# Autodesk Inventor assembly: Tower Assembly
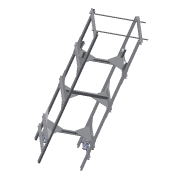
[picture p0: Inventor's stored thumbnail of the model, 180x180]
Saved by Autodesk Inventor 2015 (Build 190159000, 159)
## iProperties
Created: 2015-01-24
Part Number: Tower Assembly
Document SubType Name: Assembly
Designer: Peter
Author: Peter
## Documents named in this file (13)
- C:\Users\Noah\Desktop\FIRST-Team-1719-CAD-Team\2015 Robot CAD\Lifter Super Structure\Tower\Tower Assembly.iam
- C:\Users\Noah\Desktop\FIRST-Team-1719-CAD-Team\2015 Robot CAD\Lifter Super Structure\Tower\Side-Towers Assemblies\Left Side Tower Assembly.iam
- C:\Users\Noah\Desktop\FIRST-Team-1719-CAD-Team\2015 Robot CAD\Lifter Super Structure\Tower\Side-Towers Assemblies\Right Side Tower Assembly.iam
- C:\Users\Noah\Desktop\FIRST-Team-1719-CAD-Team\2015 Robot CAD\Lifter Super Structure\Tower\H-Shaped-Assembly\H-Shaped-Assembly.iam
- C:\Users\Noah\Desktop\FIRST-Team-1719-CAD-Team\2015 Robot CAD\Lifter Super Structure\Tower\Side-Towers Assemblies\Right Side Tower Assembly_MIR.iam
- C:\Users\Noah\Desktop\FIRST-Team-1719-CAD-Team\2015 Robot CAD\Lifter Super Structure\Tower\Side-Towers Assemblies\Left Side Tower Assembly_MIR.iam
- C:\Users\Noah\Desktop\FIRST-Team-1719-CAD-Team\2015 Robot CAD\Lifter Super Structure\Tower\Elevator Motor Assembly\Elevator Motor Assembly_MIR1.iam
- C:\Users\Noah\Desktop\FIRST-Team-1719-CAD-Team\2015 Robot CAD\Lifter Super Structure\Tower\Chain Tension\Chain Tension - L Bracket - Base.ipt
- C:\Users\Noah\Desktop\FIRST-Team-1719-CAD-Team\2015 Robot CAD\Lifter Super Structure\Tower\Chain Tension\Chain Tension - L Bracket.ipt
- C:\Users\Noah\Desktop\FIRST-Team-1719-CAD-Team\2015 Robot CAD\Lifter Super Structure\Tower\Chain Tension\pulley  pinion 1 in 16T 615378 mod1.ipt
- C:\Users\Noah\Desktop\FIRST-Team-1719-CAD-Team\2015 Robot CAD\Lifter Super Structure\Tower\H-Shaped-Assembly\Horizontal-Unistrut-Tower-Connector-15 w holes.ipt
- C:\Users\Noah\Desktop\FIRST-Team-1719-CAD-Team\2015 Robot CAD\Lifter Super Structure\Tower\Top Assembly\Tower connecter.ipt
- C:\Users\Noah\Desktop\FIRST-Team-1719-CAD-Team\2015 Robot CAD\Lifter Super Structure\Tower\Top Assembly\Tower shaft collar bearing.ipt
## Components (29 placed, 12 different names)
1. Right Side Tower Assembly:1 [sub-assembly] — Flush:9, Mate:5, Symmetry:1, Mate:10, Mate:17, Flush:19, Flush:20, Mate:30
2. Left Side Tower Assembly:1 [sub-assembly] — Mate:3, Mate:4, Flush:5, Flush:6, Flush:7, Flush:8, Flush:10, Mate:8, Mate:16, Flush:17, Flush:18, Flush:29
3. H-Shaped-Assembly:5 [sub-assembly] — Mate:3, Flush:5, Flush:8, Mate:7, Flush:13, Mate:9, Flush:14, Mate:11, Mate:12, Flush:15, Flush:16
4. H-Shaped-Assembly:6 [sub-assembly] — Mate:4, Flush:6, Flush:7, Angle:1, Angle:30
5. H-Shaped-Assembly:7 [sub-assembly] — Flush:9, Mate:5, Flush:10
6. Right Side Tower Assembly_MIR:1 [sub-assembly] — Symmetry:1, Mate:15, Flush:23, Flush:24
7. Left Side Tower Assembly_MIR:1 [sub-assembly] — Mate:13, Mate:14, Mate:18, Flush:21, Flush:22, Mate:29, Flush:27, Flush:28
8. Chain Tension - L Bracket - Base:1 — Mate:11, Mate:14, Flush:16, Insert:4
9. Chain Tension - L Bracket - Base:2 — Mate:12, Mate:13, Flush:15, Insert:3, Mate:15
10. Chain Tension - L Bracket - Base:3 — Mate:9, Flush:14, Mate:10, Insert:1
11. Chain Tension - L Bracket - Base:4 — Mate:7, Flush:13, Mate:8, Insert:2
12. Chain Tension - L Bracket:1 — Insert:1, Insert:5
13. Chain Tension - L Bracket:2 — Insert:4, Insert:8
14. Chain Tension - L Bracket:3 — Insert:2, Insert:6
15. Chain Tension - L Bracket:4 — Insert:3, Insert:7
16. pulley  pinion 1 in 16T 615378 mod1:1 — Insert:5
17. pulley  pinion 1 in 16T 615378 mod1:2 — Insert:6
18. pulley  pinion 1 in 16T 615378 mod1:3 — Insert:8
19. pulley  pinion 1 in 16T 615378 mod1:4 — Insert:7
20. Horizontal-Unistrut-Tower-Connector-15 w holes:1 — Mate:18, Flush:21, Flush:22, Flush:23, Flush:24, Flush:25, Mate:23, Mate:28
21. Horizontal-Unistrut-Tower-Connector-15 w holes:2 — Mate:16, Flush:17, Flush:18, Mate:17, Flush:19, Flush:20, Mate:20, Mate:21, Flush:26, Mate:25, Mate:26
22. Tower connecter:1 — Flush:25, Mate:19, Mate:22
23. Tower connecter:2 — Flush:26, Mate:24, Mate:27
24. Tower shaft collar bearing:1 — Mate:19, Mate:20, Mate:21
25. Tower shaft collar bearing:2 — Mate:22, Mate:23
26. Tower shaft collar bearing:3 — Mate:27, Mate:28
27. Tower shaft collar bearing:4 — Mate:24, Mate:25, Mate:26
28. Elevator Motor Assembly_MIR1:1 [sub-assembly] — Mate:29, Angle:1, Flush:27, Flush:28, Flush:30
29. Elevator Motor Assembly_MIR1:2 [sub-assembly] — Mate:30, Angle:30, Flush:29, Flush:30
## Relationships (62: Mate 27, Flush 24, Insert 8, Angle 2, Symmetry 1)
- Mate:3: Left Side Tower Assembly:1 ↔ H-Shaped-Assembly:5
- Mate:4: Left Side Tower Assembly:1 ↔ H-Shaped-Assembly:6
- Flush:5: Left Side Tower Assembly:1 ↔ H-Shaped-Assembly:5
- Flush:6: Left Side Tower Assembly:1 ↔ H-Shaped-Assembly:6
- Flush:7: Left Side Tower Assembly:1 ↔ H-Shaped-Assembly:6
- Flush:8 (-93.6625 mm): Left Side Tower Assembly:1 ↔ H-Shaped-Assembly:5
- Flush:9: Right Side Tower Assembly:1 ↔ H-Shaped-Assembly:7
- Mate:5: Right Side Tower Assembly:1 ↔ H-Shaped-Assembly:7
- Flush:10 (-93.6625 mm): Left Side Tower Assembly:1 ↔ H-Shaped-Assembly:7
- Symmetry:1: Right Side Tower Assembly:1 ↔ Right Side Tower Assembly_MIR:1
- Mate:7: H-Shaped-Assembly:5 ↔ Chain Tension - L Bracket - Base:4
- Flush:13: H-Shaped-Assembly:5 ↔ Chain Tension - L Bracket - Base:4
- Mate:8 (3.302 mm): Left Side Tower Assembly:1 ↔ Chain Tension - L Bracket - Base:4
- Mate:9: H-Shaped-Assembly:5 ↔ Chain Tension - L Bracket - Base:3
- Flush:14: H-Shaped-Assembly:5 ↔ Chain Tension - L Bracket - Base:3
- Mate:10 (3.302 mm): Right Side Tower Assembly:1 ↔ Chain Tension - L Bracket - Base:3
- Mate:11: H-Shaped-Assembly:5 ↔ Chain Tension - L Bracket - Base:1
- Mate:12: H-Shaped-Assembly:5 ↔ Chain Tension - L Bracket - Base:2
- Mate:13 (3.302 mm): Left Side Tower Assembly_MIR:1 ↔ Chain Tension - L Bracket - Base:2
- Mate:14 (3.302 mm): Left Side Tower Assembly_MIR:1 ↔ Chain Tension - L Bracket - Base:1
- Flush:15: H-Shaped-Assembly:5 ↔ Chain Tension - L Bracket - Base:2
- Flush:16: H-Shaped-Assembly:5 ↔ Chain Tension - L Bracket - Base:1
- Insert:1: Chain Tension - L Bracket - Base:3 ↔ Chain Tension - L Bracket:1
- Insert:2: Chain Tension - L Bracket - Base:4 ↔ Chain Tension - L Bracket:3
- Insert:3: Chain Tension - L Bracket - Base:2 ↔ Chain Tension - L Bracket:4
- Mate:15 (3.302 mm): Right Side Tower Assembly_MIR:1 ↔ Chain Tension - L Bracket - Base:2
- Insert:4: Chain Tension - L Bracket - Base:1 ↔ Chain Tension - L Bracket:2
- Insert:5: Chain Tension - L Bracket:1 ↔ pulley  pinion 1 in 16T 615378 mod1:1
- Insert:6: Chain Tension - L Bracket:3 ↔ pulley  pinion 1 in 16T 615378 mod1:2
- Insert:7: Chain Tension - L Bracket:4 ↔ pulley  pinion 1 in 16T 615378 mod1:4
- Insert:8: Chain Tension - L Bracket:2 ↔ pulley  pinion 1 in 16T 615378 mod1:3
- Mate:16: Left Side Tower Assembly:1 ↔ Horizontal-Unistrut-Tower-Connector-15 w holes:2
- Flush:17: Left Side Tower Assembly:1 ↔ Horizontal-Unistrut-Tower-Connector-15 w holes:2
- Flush:18: Left Side Tower Assembly:1 ↔ Horizontal-Unistrut-Tower-Connector-15 w holes:2
- Mate:17: Right Side Tower Assembly:1 ↔ Horizontal-Unistrut-Tower-Connector-15 w holes:2
- Flush:19: Right Side Tower Assembly:1 ↔ Horizontal-Unistrut-Tower-Connector-15 w holes:2
- Flush:20: Right Side Tower Assembly:1 ↔ Horizontal-Unistrut-Tower-Connector-15 w holes:2
- Mate:18: Left Side Tower Assembly_MIR:1 ↔ Horizontal-Unistrut-Tower-Connector-15 w holes:1
- Flush:21: Left Side Tower Assembly_MIR:1 ↔ Horizontal-Unistrut-Tower-Connector-15 w holes:1
- Flush:22: Left Side Tower Assembly_MIR:1 ↔ Horizontal-Unistrut-Tower-Connector-15 w holes:1
- Flush:23: Right Side Tower Assembly_MIR:1 ↔ Horizontal-Unistrut-Tower-Connector-15 w holes:1
- Flush:24: Right Side Tower Assembly_MIR:1 ↔ Horizontal-Unistrut-Tower-Connector-15 w holes:1
- Flush:25 (-88.9 mm): Horizontal-Unistrut-Tower-Connector-15 w holes:1 ↔ Tower connecter:1
- Mate:19: Tower connecter:1 ↔ Tower shaft collar bearing:1
- Mate:20: Horizontal-Unistrut-Tower-Connector-15 w holes:2 ↔ Tower shaft collar bearing:1
- Mate:21: Horizontal-Unistrut-Tower-Connector-15 w holes:2 ↔ Tower shaft collar bearing:1
- Mate:22: Tower connecter:1 ↔ Tower shaft collar bearing:2
- Mate:23: Horizontal-Unistrut-Tower-Connector-15 w holes:1 ↔ Tower shaft collar bearing:2
- Flush:26 (-38.1 mm): Horizontal-Unistrut-Tower-Connector-15 w holes:2 ↔ Tower connecter:2
- Mate:24: Tower connecter:2 ↔ Tower shaft collar bearing:4
- Mate:25: Horizontal-Unistrut-Tower-Connector-15 w holes:2 ↔ Tower shaft collar bearing:4
- Mate:26: Horizontal-Unistrut-Tower-Connector-15 w holes:2 ↔ Tower shaft collar bearing:4
- Mate:27: Tower connecter:2 ↔ Tower shaft collar bearing:3
- Mate:28: Horizontal-Unistrut-Tower-Connector-15 w holes:1 ↔ Tower shaft collar bearing:3
- Mate:29: Left Side Tower Assembly_MIR:1 ↔ Elevator Motor Assembly_MIR1:1
- Angle:1 (0 deg): H-Shaped-Assembly:6 ↔ Elevator Motor Assembly_MIR1:1
- Flush:27: Left Side Tower Assembly_MIR:1 ↔ Elevator Motor Assembly_MIR1:1
- Flush:28 (165.1 mm): Left Side Tower Assembly_MIR:1 ↔ Elevator Motor Assembly_MIR1:1
- Mate:30: Right Side Tower Assembly:1 ↔ Elevator Motor Assembly_MIR1:2
- Angle:30 (0 deg): H-Shaped-Assembly:6 ↔ Elevator Motor Assembly_MIR1:2
- Flush:29: Left Side Tower Assembly:1 ↔ Elevator Motor Assembly_MIR1:2
- Flush:30: Elevator Motor Assembly_MIR1:1 ↔ Elevator Motor Assembly_MIR1:2
